# Autodesk Inventor assembly: ClawPart
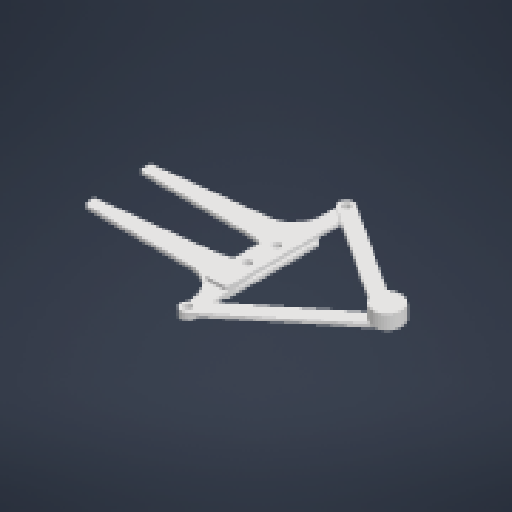
[picture p0: Inventor's stored thumbnail of the model, 512x512]
Saved by Autodesk Inventor 2023 (Build 270158000, 158)
## iProperties
Created: 2023-01-27
Part Number: ClawPart
Document SubType Name: Assembly
Designer: Terrence
Author: Terrence
## Documents named in this file (5)
- C:\Users\Terrence\Documents\FRC Long\ClawPart.iam
- C:\Users\Terrence\Documents\FRC Long\Solid1.ipt
- C:\Users\Terrence\Documents\FRC Long\Solid2.ipt
- C:\Users\Terrence\Documents\FRC Long\Solid3.ipt
- C:\Users\Terrence\Documents\FRC Long\CIR4CLE.ipt
## Components (7 placed, 4 different names)
1. Solid1:1 — Insert:1, Insert:2, Insert:3
2. Solid2:1 — Insert:1, Insert:5
3. Solid3:1 — Insert:2, Insert:7
4. Solid2:2 — Insert:3, Insert:4
5. Solid1:2 — Insert:4, Insert:5, Insert:6
6. Solid3:2 — Insert:6, Insert:7, Insert:8
7. CIR4CLE:1 — Insert:8
## Relationships (8: Insert 8)
- Insert:1: Solid1:1 ↔ Solid2:1
- Insert:2: Solid1:1 ↔ Solid3:1
- Insert:3: Solid1:1 ↔ Solid2:2
- Insert:4: Solid2:2 ↔ Solid1:2
- Insert:5: Solid2:1 ↔ Solid1:2
- Insert:6: Solid1:2 ↔ Solid3:2
- Insert:7: Solid3:1 ↔ Solid3:2
- Insert:8: Solid3:2 ↔ CIR4CLE:1
